# Autodesk Inventor assembly: 2
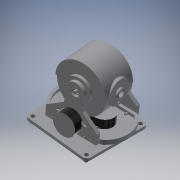
[picture p0: Inventor's stored thumbnail of the model, 180x180]
Saved by Autodesk Inventor 2018 (Build 220112000, 112)
## iProperties
Created: 2018-04-27
Part Number: 2
Material: 일반
Document SubType Name: Assembly
Designer: CK
Author: CK
## Documents named in this file (9)
- C:\Users\CK\Desktop\캡스톤\2.iam
- C:\Users\CK\Desktop\캡스톤\밑판(new).ipt
- C:\Users\CK\Desktop\캡스톤\탑(모터쪽옆면수정).ipt
- C:\Users\CK\Desktop\캡스톤\탑(옆면수정).ipt
- C:\Users\CK\Desktop\캡스톤\연결부.ipt
- C:\Users\CK\Desktop\캡스톤\큰 기어.ipt
- C:\Users\CK\Desktop\캡스톤\스텝모터.ipt
- C:\Users\CK\Desktop\캡스톤\헤드(상).ipt
- C:\Users\CK\Desktop\캡스톤\헤드(하).ipt
## Components (9 placed, 8 different names)
1. 밑판(new):1 — 메이트:1, 메이트:2, 메이트:3, 메이트:4, 메이트:5, 메이트:6, 메이트:7, 메이트:8, 메이트:9, 메이트:16, 메이트:17
2. 탑(모터쪽옆면수정):1 — 메이트:1, 메이트:2, 메이트:10, 메이트:11, 메이트:12, 메이트:14, 메이트:17
3. 탑(옆면수정):1 — 메이트:3, 메이트:4, 메이트:15, 메이트:16
4. 연결부:1 — 삽입:1, 메이트:13
5. 큰 기어:1 — 메이트:5, 메이트:6, 삽입:1
6. 스텝모터:1 — 메이트:10, 메이트:11, 메이트:12
7. 스텝모터:2 — 메이트:7, 메이트:8, 메이트:9
8. 헤드(상):1 — 메이트:14, 메이트:15, 메이트:21, 메이트:22, 메이트:23
9. 헤드(하):1 — 메이트:21, 메이트:22, 메이트:23
## Relationships (21: Mate 20, Insert 1)
- 메이트:1 [Mate]: 밑판(new):1 ↔ 탑(모터쪽옆면수정):1
- 메이트:2 [Mate]: 밑판(new):1 ↔ 탑(모터쪽옆면수정):1
- 메이트:3 [Mate]: 밑판(new):1 ↔ 탑(옆면수정):1
- 메이트:4 [Mate]: 밑판(new):1 ↔ 탑(옆면수정):1
- 메이트:5 [Mate]: 밑판(new):1 ↔ 큰 기어:1
- 메이트:6 [Mate]: 밑판(new):1 ↔ 큰 기어:1
- 메이트:7 [Mate]: 밑판(new):1 ↔ 스텝모터:2
- 메이트:8 [Mate]: 밑판(new):1 ↔ 스텝모터:2
- 메이트:9 [Mate]: 밑판(new):1 ↔ 스텝모터:2
- 메이트:10 [Mate]: 탑(모터쪽옆면수정):1 ↔ 스텝모터:1
- 메이트:11 [Mate]: 탑(모터쪽옆면수정):1 ↔ 스텝모터:1
- 메이트:12 [Mate]: 탑(모터쪽옆면수정):1 ↔ 스텝모터:1
- 삽입:1 [Insert]: 연결부:1 ↔ 큰 기어:1
- 메이트:13 [Mate]: 연결부:1
- 메이트:14 [Mate]: 탑(모터쪽옆면수정):1 ↔ 헤드(상):1
- 메이트:15 [Mate]: 탑(옆면수정):1 ↔ 헤드(상):1
- 메이트:16 [Mate]: 밑판(new):1 ↔ 탑(옆면수정):1
- 메이트:17 [Mate]: 밑판(new):1 ↔ 탑(모터쪽옆면수정):1
- 메이트:21 [Mate]: 헤드(상):1 ↔ 헤드(하):1
- 메이트:22 [Mate]: 헤드(상):1 ↔ 헤드(하):1
- 메이트:23 [Mate]: 헤드(상):1 ↔ 헤드(하):1
